# Autodesk Inventor assembly: Мостики
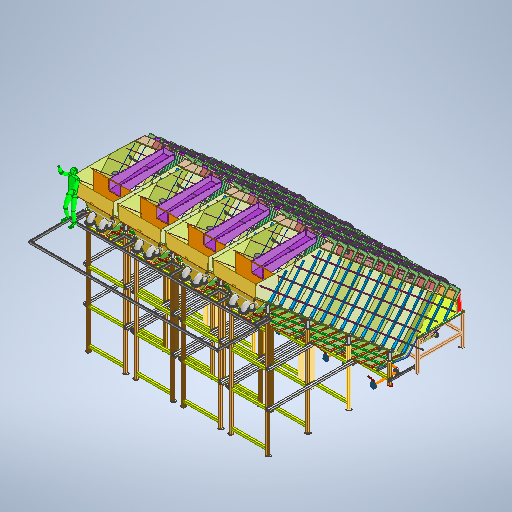
[picture p0: Inventor's stored thumbnail of the model, 512x512]
Saved by Autodesk Inventor 2025 (Build 290162010, 162A)
## iProperties
Created: 2025-01-27
Part Number: Мостики
Document SubType Name: Assembly
Designer: admin
Author: admin
## Documents named in this file (4)
- C:\Users\pokla\Documents\Inventor\Отстойник осветлитель\Manturovo_Se-clar-Gleb\Мостики.iam
- C:\Users\pokla\Documents\Inventor\Отстойник осветлитель\Manturovo_Se-clar-Gleb\ASY MSC 002 отстойник осветлитель.iam
- C:\Users\pokla\Documents\Inventor\Отстойник осветлитель\Manturovo_Se-clar-Gleb\human 01\ч ASY human dummy 01.iam
- C:\Users\pokla\Documents\Inventor\Отстойник осветлитель\Manturovo_Se-clar-Gleb\ASY MSC Платформа отстойников.iam
## Components (6 placed, 3 different names)
1. ASY MSC 002 отстойник осветлитель:1 [sub-assembly] — Flush:1, Flush:2, Flush:3, Flush:4, Rigid:1, Flush:5, Mate:1
2. ASY MSC 002 отстойник осветлитель:2 [sub-assembly] — Rigid:1, Rigid:2
3. ASY MSC 002 отстойник осветлитель:3 [sub-assembly] — Rigid:3
4. ASY MSC 002 отстойник осветлитель:4 [sub-assembly] — Rigid:2, Rigid:3
5. ч ASY human dummy 01:1 [sub-assembly] — Flush:1
6. ASY MSC Платформа отстойников:1 [sub-assembly] — Flush:5, Mate:1, Mate:2
## Relationships (10: Flush 5, WeldJoint 3, Mate 2)
- Flush:1 (4500 mm): ASY MSC 002 отстойник осветлитель:1 ↔ ч ASY human dummy 01:1
- Flush:2: ASY MSC 002 отстойник осветлитель:1
- Flush:3: ASY MSC 002 отстойник осветлитель:1
- Flush:4: ASY MSC 002 отстойник осветлитель:1
- Rigid:1 [WeldJoint] (50 mm): ASY MSC 002 отстойник осветлитель:1 ↔ ASY MSC 002 отстойник осветлитель:2
- Rigid:2 [WeldJoint] (50 mm): ASY MSC 002 отстойник осветлитель:2 ↔ ASY MSC 002 отстойник осветлитель:4
- Rigid:3 [WeldJoint] (50 mm): ASY MSC 002 отстойник осветлитель:3 ↔ ASY MSC 002 отстойник осветлитель:4
- Flush:5: ASY MSC 002 отстойник осветлитель:1 ↔ ASY MSC Платформа отстойников:1
- Mate:1: ASY MSC 002 отстойник осветлитель:1 ↔ ASY MSC Платформа отстойников:1
- Mate:2 (4400 mm): ASY MSC Платформа отстойников:1
